# Autodesk Inventor assembly: NUEVO Ensamble de estructura H
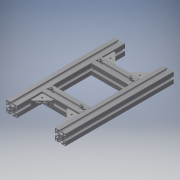
[picture p0: Inventor's stored thumbnail of the model, 180x180]
Saved by Autodesk Inventor 2018.3 (Build 223284000, 284)
## iProperties
Created: 2020-12-03
Part Number: NUEVO Ensamble de estructura H
Material: Genérico
Description: STEP AP203
Document SubType Name: Assembly
Designer: SERGIO ROMO
Sending System: SolidWorks 2019
Preprocessor: SwSTEP 2.0
Title: Ensamble del Arreglo.STEP
Revision Number: ANY
## Documents named in this file (8)
- C:\Users\SERGIO ROMO\Documents\GitHub\RemBot\CAD\Balanceo de masa\Inventor\NUEVO Ensamble de estructura H.iam
- C:\Users\SERGIO ROMO\Documents\GitHub\RemBot\CAD\Balanceo de masa\Inventor\Perfil de Aluminio.ipt
- C:\Users\SERGIO ROMO\Documents\GitHub\RemBot\CAD\Balanceo de masa\Inventor\Perfil de Aluminio corta.ipt
- C:\Users\SERGIO ROMO\Documents\GitHub\RemBot\CAD\Balanceo de masa\Inventor\TornilloM6.ipt
- C:\Users\SERGIO ROMO\Documents\GitHub\RemBot\CAD\Balanceo de masa\Inventor\Tuerca para tornilloM6.ipt
- C:\Users\SERGIO ROMO\Documents\GitHub\RemBot\CAD\Balanceo de masa\Inventor\Sujetador.ipt
- C:\Users\SERGIO ROMO\Documents\GitHub\RemBot\CAD\Balanceo de masa\Inventor\TornilloM8.ipt
- C:\Users\SERGIO ROMO\Documents\GitHub\RemBot\CAD\Balanceo de masa\Inventor\Tuerca para tornilloM8.ipt
## Components (32 placed, 8 different names)
1. Perfil de Aluminio_4 — Coincidencia:37, Coincidencia:60, Coincidencia:61, Coincidencia:75, Coincidencia:77
2. Perfil de Aluminio_5 — Coincidencia:36, Coincidencia:64, Coincidencia:66, Coincidencia:79, Coincidencia:81
3. Perfil de Aluminio corta:1 — Coincidencia:37, Coincidencia:46, Coincidencia:55, Coincidencia:62, Coincidencia:63, Coincidencia:71, Coincidencia:72
4. Perfil de Aluminio corta:2 — Coincidencia:36, Coincidencia:51, Coincidencia:56, Coincidencia:59, Coincidencia:65, Coincidencia:67, Coincidencia:68
5. TornilloM6:1 — Coincidencia:46, Coincidencia:48
6. Tuerca para tornilloM6:1 — Coincidencia:48
7. TornilloM6:2 — Coincidencia:51, Coincidencia:52
8. Tuerca para tornilloM6:2 — Coincidencia:52
9. TornilloM6:3 — Coincidencia:56, Coincidencia:57
10. TornilloM6:4 — Coincidencia:55, Coincidencia:58
11. Tuerca para tornilloM6:3 — Coincidencia:57
12. Tuerca para tornilloM6:4 — Coincidencia:58
13. Sujetador:1 — Coincidencia:59, Coincidencia:60
14. Sujetador:2 — Coincidencia:61, Coincidencia:62
15. Sujetador:3 — Coincidencia:65, Coincidencia:66
16. Sujetador:4 — Coincidencia:63, Coincidencia:64
17. TornilloM8:1 — Coincidencia:68, Coincidencia:70
18. TornilloM8:2 — Coincidencia:67, Coincidencia:69
19. Tuerca para tornilloM8:1 — Coincidencia:69
20. Tuerca para tornilloM8:2 — Coincidencia:70
21. TornilloM8:3 — Coincidencia:71, Coincidencia:74
22. TornilloM8:4 — Coincidencia:72, Coincidencia:73
23. Tuerca para tornilloM8:3 — Coincidencia:73
24. Tuerca para tornilloM8:4 — Coincidencia:74
25. TornilloM8:5 — Coincidencia:75, Coincidencia:76
26. TornilloM8:6 — Coincidencia:77, Coincidencia:78
27. Tuerca para tornilloM8:5 — Coincidencia:76
28. Tuerca para tornilloM8:6 — Coincidencia:78
29. TornilloM8:7 — Coincidencia:81, Coincidencia:82
30. TornilloM8:8 — Coincidencia:79, Coincidencia:80
31. Tuerca para tornilloM8:7 — Coincidencia:80
32. Tuerca para tornilloM8:8 — Coincidencia:82
## Relationships (34: Mate 34)
- Coincidencia:36 [Mate]: Perfil de Aluminio_5 ↔ Perfil de Aluminio corta:2
- Coincidencia:37 [Mate]: Perfil de Aluminio_4 ↔ Perfil de Aluminio corta:1
- Coincidencia:46 [Mate]: Perfil de Aluminio corta:1 ↔ TornilloM6:1
- Coincidencia:48 [Mate]: TornilloM6:1 ↔ Tuerca para tornilloM6:1
- Coincidencia:51 [Mate]: Perfil de Aluminio corta:2 ↔ TornilloM6:2
- Coincidencia:52 [Mate]: TornilloM6:2 ↔ Tuerca para tornilloM6:2
- Coincidencia:55 [Mate]: Perfil de Aluminio corta:1 ↔ TornilloM6:4
- Coincidencia:56 [Mate]: Perfil de Aluminio corta:2 ↔ TornilloM6:3
- Coincidencia:57 [Mate]: TornilloM6:3 ↔ Tuerca para tornilloM6:3
- Coincidencia:58 [Mate]: TornilloM6:4 ↔ Tuerca para tornilloM6:4
- Coincidencia:59 [Mate]: Perfil de Aluminio corta:2 ↔ Sujetador:1
- Coincidencia:60 [Mate]: Perfil de Aluminio_4 ↔ Sujetador:1
- Coincidencia:61 [Mate]: Perfil de Aluminio_4 ↔ Sujetador:2
- Coincidencia:62 [Mate]: Perfil de Aluminio corta:1 ↔ Sujetador:2
- Coincidencia:63 [Mate]: Perfil de Aluminio corta:1 ↔ Sujetador:4
- Coincidencia:64 [Mate]: Perfil de Aluminio_5 ↔ Sujetador:4
- Coincidencia:65 [Mate]: Perfil de Aluminio corta:2 ↔ Sujetador:3
- Coincidencia:66 [Mate]: Perfil de Aluminio_5 ↔ Sujetador:3
- Coincidencia:67 [Mate]: Perfil de Aluminio corta:2 ↔ TornilloM8:2
- Coincidencia:68 [Mate]: Perfil de Aluminio corta:2 ↔ TornilloM8:1
- Coincidencia:69 [Mate]: TornilloM8:2 ↔ Tuerca para tornilloM8:1
- Coincidencia:70 [Mate]: TornilloM8:1 ↔ Tuerca para tornilloM8:2
- Coincidencia:71 [Mate]: Perfil de Aluminio corta:1 ↔ TornilloM8:3
- Coincidencia:72 [Mate]: Perfil de Aluminio corta:1 ↔ TornilloM8:4
- Coincidencia:73 [Mate]: TornilloM8:4 ↔ Tuerca para tornilloM8:3
- Coincidencia:74 [Mate]: TornilloM8:3 ↔ Tuerca para tornilloM8:4
- Coincidencia:75 [Mate]: Perfil de Aluminio_4 ↔ TornilloM8:5
- Coincidencia:76 [Mate]: TornilloM8:5 ↔ Tuerca para tornilloM8:5
- Coincidencia:77 [Mate]: Perfil de Aluminio_4 ↔ TornilloM8:6
- Coincidencia:78 [Mate]: TornilloM8:6 ↔ Tuerca para tornilloM8:6
- Coincidencia:79 [Mate]: Perfil de Aluminio_5 ↔ TornilloM8:8
- Coincidencia:80 [Mate]: TornilloM8:8 ↔ Tuerca para tornilloM8:7
- Coincidencia:81 [Mate]: Perfil de Aluminio_5 ↔ TornilloM8:7
- Coincidencia:82 [Mate]: TornilloM8:7 ↔ Tuerca para tornilloM8:8
